# Autodesk Inventor assembly: baseWithWormGearAndLock
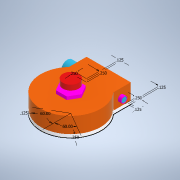
[picture p0: Inventor's stored thumbnail of the model, 180x180]
Saved by Autodesk Inventor 2021.2 (Build 252289000, 289)
## iProperties
Created: 2020-11-22
Part Number: baseWithWormGearAndLock
Document SubType Name: Assembly
Designer: robst
Author: robst
## Documents named in this file (14)
- C:\git\CAD-Development\robSteele\ShapeWays\TelescopeProjects\TelescopeMountNov2020\baseWithWormGearAndLock.iam
- C:\git\CAD-Development\robSteele\ShapeWays\TelescopeProjects\TelescopeMountNov2020\baseSupport.ipt
- C:\git\CAD-Development\robSteele\ShapeWays\TelescopeProjects\TelescopeMountNov2020\3_8x4_5-inchHexShaft.ipt
- C:\git\CAD-Development\robSteele\ShapeWays\TelescopeProjects\TelescopeMountNov2020\3_8x5_8x3_4-hexBearing.ipt
- C:\git\CAD-Development\robSteele\ShapeWays\TelescopeProjects\TelescopeMountNov2020\3_8x5_8x3_4-hexBearingEndCap.ipt
- C:\git\CAD-Development\robSteele\ShapeWays\TelescopeProjects\TelescopeMountNov2020\1_2x3-inchHexShaft.ipt
- C:\git\CAD-Development\robSteele\ShapeWays\TelescopeProjects\TelescopeMountNov2020\1_2x1-hexBushing.ipt
- C:\git\CAD-Development\robSteele\ShapeWays\TelescopeProjects\TelescopeMount\forkMountForDecTripV01\Design Accelerator\Worm Gears5.iam
- C:\git\CAD-Development\robSteele\ShapeWays\TelescopeProjects\TelescopeMountNov2020\1_2x2x3_16-hexBearing.ipt
- C:\git\CAD-Development\robSteele\ShapeWays\TelescopeProjects\TelescopeMountNov2020\gearLock.ipt
- C:\git\CAD-Development\robSteele\ShapeWays\TelescopeProjects\TelescopeMountNov2020\baseSupportCover.ipt
- C:\Users\robst\Documents\Inventor\Content Center Files\R2021\en-US\ANSI B18.22.1\ANSI B18.22.1 - No. 6 - narrow - Type B.ipt
- C:\Users\robst\Documents\Inventor\Content Center Files\R2021\en-US\ASME B18.21.1(10)\ASME B18.21.1 - No.6(2).ipt
- C:\Users\robst\Documents\Inventor\Content Center Files\R2021\en-US\ANSI B18.3(11)\ANSI B18.3 - 6-32 UNC - 1.5(23).ipt
## Components (13 placed, 13 different names)
1. baseSupport:1 — Insert:1, Insert:3, Insert:4, Insert:5, Mate:1, Flush:1, Flush:2
2. 3_8x4_5-inchHexShaft:1 — Insert:1, Insert:2
3. 3_8x5_8x3_4-hexBearing:1 — Insert:2
4. 3_8x5_8x3_4-hexBearingEndCap:1 — Insert:3
5. 1_2x3-inchHexShaft:1 — Insert:4
6. 1_2x1-hexBushing:1 — Insert:5, Insert:6
7. Worm Gears:1 [sub-assembly] — Insert:6, Insert:7
8. 1_2x2x3_16-hexBearing:1 — Insert:7, Insert:8
9. gearLock:1 — Insert:8
10. baseSupportCover:1 — Mate:1, Flush:1, Flush:2
11. Plain Washer (Inch) No. 6 - narrow - Type B:1
12. Regular Helical Spring Lock Washer (Inch) No.6:1
13. Spline Socket Button Head Cap Screw - Inch 6-32 UNC - 1.5:1
## Relationships (11: Insert 8, Flush 2, Mate 1)
- Insert:1: baseSupport:1 ↔ 3_8x4_5-inchHexShaft:1
- Insert:2: 3_8x4_5-inchHexShaft:1 ↔ 3_8x5_8x3_4-hexBearing:1
- Insert:3: baseSupport:1 ↔ 3_8x5_8x3_4-hexBearingEndCap:1
- Insert:4 (12.7 mm): baseSupport:1 ↔ 1_2x3-inchHexShaft:1
- Insert:5: baseSupport:1 ↔ 1_2x1-hexBushing:1
- Insert:6: 1_2x1-hexBushing:1 ↔ Worm Gears:1
- Insert:7: Worm Gears:1 ↔ 1_2x2x3_16-hexBearing:1
- Insert:8: 1_2x2x3_16-hexBearing:1 ↔ gearLock:1
- Mate:1: baseSupport:1 ↔ baseSupportCover:1
- Flush:1: baseSupport:1 ↔ baseSupportCover:1
- Flush:2: baseSupport:1 ↔ baseSupportCover:1
